# Autodesk Inventor assembly: A2017_T4_01
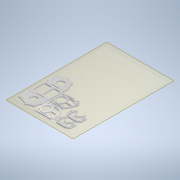
[picture p0: Inventor's stored thumbnail of the model, 180x180]
Saved by Autodesk Inventor 2020 (Build 240168000, 168)
## iProperties
Created: 2021-08-27
Part Number: A2017_T4_01
Document SubType Name: Assembly
Designer: Masato
Author: Masato
## Documents named in this file (6)
- C:\Users\naoki\Documents\Inventor\CitBrains\git_clone\OpenPlatform4_0\CAM\A2017_T4_肩修正後\OpenPlatform_ver3_0\cam\A2017_T4_01.iam
- C:\Users\naoki\Documents\Inventor\CitBrains\git_clone\OpenPlatform4_0\CAM\A2017_T4_肩修正後\OpenPlatform_ver3_0\cam\Disposable_Board.ipt
- C:\Users\naoki\Documents\Inventor\CitBrains\git_clone\OpenPlatform4_0\CAM\A2017_T4_肩修正後\OpenPlatform_ver3_0\UpperBody\Trunk\Trunk_lower_waisit_frame.ipt
- C:\Users\naoki\Documents\Inventor\CitBrains\git_clone\OpenPlatform4_0\CAM\A2017_T4_肩修正後\OpenPlatform_ver3_0\UpperBody\Trunk\Trunk_shoulder_frame.ipt
- C:\Users\naoki\Documents\Inventor\CitBrains\git_clone\OpenPlatform4_0\CAM\A2017_T4_肩修正後\OpenPlatform_ver3_0\UpperBody\Trunk\Trunk_shoulder_frame_MIR.ipt
- C:\Users\naoki\Documents\Inventor\CitBrains\git_clone\OpenPlatform4_0\CAM\A2017_T4_肩修正後\OpenPlatform_ver3_0\LowerBody\Leg_joit\Leg_joint_roll_back_frame.ipt
## Components (6 placed, 5 different names)
1. Disposable_Board:1 — メイト:2, メイト:1, フラッシュ:1, フラッシュ:2, メイト:5, 正接:1, フラッシュ:5
2. Trunk_lower_waisit_frame:1 — メイト:6, 正接:1, メイト:10, フラッシュ:5, 正接:2
3. Trunk_shoulder_frame:1 — メイト:5, メイト:9, メイト:10, フラッシュ:4
4. Trunk_shoulder_frame_MIR:1 — メイト:4, フラッシュ:3, メイト:9, フラッシュ:4, 正接:2, 正接:3
5. Leg_joint_roll_back_frame:1 — メイト:8, フラッシュ:3, 正接:3
6. Leg_joint_roll_back_frame:2
## Component patterns: (2 elements, first: Leg_joint_roll_back_frame:1)
## Relationships (16: Mate 8, Flush 5, Tangent 3)
- メイト:2 [Mate]: Disposable_Board:1
- メイト:1 [Mate]: Disposable_Board:1
- フラッシュ:1 [Flush]: Disposable_Board:1
- フラッシュ:2 [Flush]: Disposable_Board:1
- メイト:4 [Mate]: Trunk_shoulder_frame_MIR:1
- メイト:5 [Mate]: Disposable_Board:1 ↔ Trunk_shoulder_frame:1
- メイト:6 [Mate]: Trunk_lower_waisit_frame:1
- メイト:8 [Mate]: Leg_joint_roll_back_frame:1
- フラッシュ:3 [Flush]: Trunk_shoulder_frame_MIR:1 ↔ Leg_joint_roll_back_frame:1
- 正接:1 [Tangent] (2 mm): Disposable_Board:1 ↔ Trunk_lower_waisit_frame:1
- メイト:9 [Mate] (2.5 mm): Trunk_shoulder_frame:1 ↔ Trunk_shoulder_frame_MIR:1
- メイト:10 [Mate] (2.5 mm): Trunk_lower_waisit_frame:1 ↔ Trunk_shoulder_frame:1
- フラッシュ:4 [Flush]: Trunk_shoulder_frame:1 ↔ Trunk_shoulder_frame_MIR:1
- フラッシュ:5 [Flush] (2 mm): Disposable_Board:1 ↔ Trunk_lower_waisit_frame:1
- 正接:2 [Tangent]: Trunk_lower_waisit_frame:1 ↔ Trunk_shoulder_frame_MIR:1
- 正接:3 [Tangent] (2.5 mm): Trunk_shoulder_frame_MIR:1 ↔ Leg_joint_roll_back_frame:1
